# Autodesk Inventor assembly: Robot
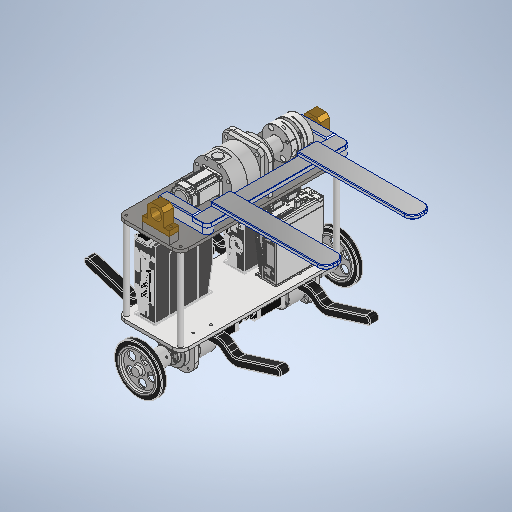
[picture p0: Inventor's stored thumbnail of the model, 512x512]
Saved by Autodesk Inventor 2025.2 (Build 292293000, 293)
## iProperties
Created: 2025-02-20
Part Number: Robot
Document SubType Name: Assembly
Designer: Sergio Quintero
Author: Sergio Quintero
## Documents named in this file (19)
- C:\Users\Sergio Quintero\OneDrive - Universidad Nacional de Colombia\Keio University\Thesis\CAD\Current\Robot.iam
- C:\Users\Sergio Quintero\OneDrive - Universidad Nacional de Colombia\Keio University\Thesis\CAD\Current\Bottom_plate.ipt
- C:\Users\Sergio Quintero\OneDrive - Universidad Nacional de Colombia\Keio University\Thesis\CAD\Current\Top_plate.ipt
- C:\Users\Sergio Quintero\OneDrive - Universidad Nacional de Colombia\Keio University\Thesis\CAD\Current\Structure_bar.ipt
- C:\Users\Sergio Quintero\OneDrive - Universidad Nacional de Colombia\Keio University\Thesis\CAD\Current\Pillow_support.ipt
- C:\Users\Sergio Quintero\OneDrive - Universidad Nacional de Colombia\Keio University\Thesis\CAD\Current\Pillow_block.ipt
- C:\Users\Sergio Quintero\OneDrive - Universidad Nacional de Colombia\Keio University\Thesis\CAD\Current\Gear_support.ipt
- C:\Users\Sergio Quintero\OneDrive - Universidad Nacional de Colombia\Keio University\Thesis\CAD\Current\HPG-32A-33-J2NELA.iam
- C:\Users\Sergio Quintero\OneDrive - Universidad Nacional de Colombia\Keio University\Thesis\CAD\Current\SFC-090SA2-25B-40B.ipt
- C:\Users\Sergio Quintero\OneDrive - Universidad Nacional de Colombia\Keio University\Thesis\CAD\Current\Fork.ipt
- C:\Users\Sergio Quintero\OneDrive - Universidad Nacional de Colombia\Keio University\Thesis\CAD\Current\Gear_support_wheel.ipt
- C:\Users\Sergio Quintero\OneDrive - Universidad Nacional de Colombia\Keio University\Thesis\CAD\Current\HPG-20A-11-J6GDK.iam
- C:\Users\Sergio Quintero\OneDrive - Universidad Nacional de Colombia\Keio University\Thesis\CAD\Current\MRG-50-25-25.ipt
- C:\Users\Sergio Quintero\OneDrive - Universidad Nacional de Colombia\Keio University\Thesis\CAD\Current\Wheel.ipt
- C:\Users\Sergio Quintero\OneDrive - Universidad Nacional de Colombia\Keio University\Thesis\CAD\Current\R88M_K40030S.ipt
- C:\Users\Sergio Quintero\OneDrive - Universidad Nacional de Colombia\Keio University\Thesis\CAD\Current\R88M_1M40030S_S2.ipt
- C:\Users\Sergio Quintero\OneDrive - Universidad Nacional de Colombia\Keio University\Thesis\CAD\Current\Robot_support.ipt
- C:\Users\Sergio Quintero\OneDrive - Universidad Nacional de Colombia\Keio University\Thesis\CAD\Current\R88D_1SN04L_ECT\R88D_1SN04L_ECT.iam
- C:\Users\Sergio Quintero\OneDrive - Universidad Nacional de Colombia\Keio University\Thesis\CAD\Current\R88D_KN04L_ECT\R88D_KN04L_ECT.iam
## Components (32 placed, 18 different names)
1. Bottom_plate:1 — Rigid:1, Rigid:2, Rigid:3, Rigid:4, Rigid:5, Rigid:13, Rigid:14, Angle:1, Rigid:23, Rigid:24, Rigid:25, Rigid:26, Rigid:27, Rigid:28, Rigid:29
2. Top_plate:1 — Rigid:5, Rigid:6, Rigid:8, Rigid:10
3. Structure_bar:1 — Rigid:4
4. Structure_bar:2 — Rigid:3
5. Structure_bar:3 — Rigid:2
6. Structure_bar:4 — Rigid:1
7. Pillow_support:1 — Rigid:6, Rigid:7
8. Pillow_block:1 — Rigid:7
9. Pillow_block:2 — Rigid:9, Rotational:1
10. Pillow_support:2 — Rigid:8, Rigid:9
11. Gear_support:1 — Rigid:10, Rigid:11
12. HPG-32A-33-J2NELA:1 [sub-assembly] — Rigid:11, Rigid:12, Rigid:21
13. SFC-090SA2-25B-40B:1 — Rigid:12
14. Fork:1 — Rotational:1
15. Gear_support_wheel:1 — Rigid:14, Rigid:15
16. Gear_support_wheel:2 — Rigid:13, Rigid:16
17. HPG-20A-11-J6GDK:1 [sub-assembly] — Rigid:15, Rigid:18, Rotational:2
18. HPG-20A-11-J6GDK:2 [sub-assembly] — Rigid:16, Rigid:17, Rigid:22
19. MRG-50-25-25:1 — Rigid:17, Rigid:20
20. MRG-50-25-25:2 — Rigid:18, Rigid:19
21. Wheel:1 — Rigid:20
22. Wheel:2 — Rigid:19, Tangent:1
23. R88M_K40030S:1 — Rigid:21
24. R88M_1M40030S_S2:1 — Rigid:22
25. R88M_1M40030S_S2:2 — Rotational:2
26. Robot_support:1 — Rigid:23
27. Robot_support:2 — Rigid:24
28. Robot_support:3 — Rigid:25
29. Robot_support:4 — Rigid:26
30. R88D_1SN04L_ECT:1 [sub-assembly] — Rigid:27
31. R88D_1SN04L_ECT:2 [sub-assembly] — Rigid:28
32. R88D_KN04L_ECT:1 [sub-assembly] — Rigid:29
## Relationships (33: WeldJoint 29, RevoluteJoint 2, Angle 1, Tangent 1)
- Rigid:1 [WeldJoint]: Bottom_plate:1 ↔ Structure_bar:4
- Rigid:2 [WeldJoint]: Bottom_plate:1 ↔ Structure_bar:3
- Rigid:3 [WeldJoint]: Bottom_plate:1 ↔ Structure_bar:2
- Rigid:4 [WeldJoint]: Bottom_plate:1 ↔ Structure_bar:1
- Rigid:5 [WeldJoint] (260 mm): Bottom_plate:1 ↔ Top_plate:1
- Rigid:6 [WeldJoint]: Top_plate:1 ↔ Pillow_support:1
- Rigid:7 [WeldJoint]: Pillow_support:1 ↔ Pillow_block:1
- Rigid:8 [WeldJoint]: Top_plate:1 ↔ Pillow_support:2
- Rigid:9 [WeldJoint]: Pillow_block:2 ↔ Pillow_support:2
- Rigid:10 [WeldJoint]: Top_plate:1 ↔ Gear_support:1
- Rigid:11 [WeldJoint]: Gear_support:1 ↔ HPG-32A-33-J2NELA:1
- Rigid:12 [WeldJoint] (50 mm): HPG-32A-33-J2NELA:1 ↔ SFC-090SA2-25B-40B:1
- Rotational:1 [RevoluteJoint] (5 mm): Pillow_block:2 ↔ Fork:1
- Rigid:13 [WeldJoint]: Bottom_plate:1 ↔ Gear_support_wheel:2
- Rigid:14 [WeldJoint]: Bottom_plate:1 ↔ Gear_support_wheel:1
- Rigid:15 [WeldJoint]: Gear_support_wheel:1 ↔ HPG-20A-11-J6GDK:1
- Rigid:16 [WeldJoint]: Gear_support_wheel:2 ↔ HPG-20A-11-J6GDK:2
- Rigid:17 [WeldJoint] (15 mm): HPG-20A-11-J6GDK:2 ↔ MRG-50-25-25:1
- Rigid:18 [WeldJoint] (15 mm): HPG-20A-11-J6GDK:1 ↔ MRG-50-25-25:2
- Rigid:19 [WeldJoint] (3 mm): MRG-50-25-25:2 ↔ Wheel:2
- Rigid:20 [WeldJoint] (3 mm): MRG-50-25-25:1 ↔ Wheel:1
- Rigid:21 [WeldJoint]: HPG-32A-33-J2NELA:1 ↔ R88M_K40030S:1
- Rigid:22 [WeldJoint]: HPG-20A-11-J6GDK:2 ↔ R88M_1M40030S_S2:1
- Rotational:2 [RevoluteJoint]: HPG-20A-11-J6GDK:1 ↔ R88M_1M40030S_S2:2
- Angle:1 (0 deg): Bottom_plate:1
- Tangent:1: Wheel:2
- Rigid:23 [WeldJoint]: Bottom_plate:1 ↔ Robot_support:1
- Rigid:24 [WeldJoint]: Bottom_plate:1 ↔ Robot_support:2
- Rigid:25 [WeldJoint]: Bottom_plate:1 ↔ Robot_support:3
- Rigid:26 [WeldJoint]: Bottom_plate:1 ↔ Robot_support:4
- Rigid:27 [WeldJoint]: Bottom_plate:1 ↔ R88D_1SN04L_ECT:1
- Rigid:28 [WeldJoint]: Bottom_plate:1 ↔ R88D_1SN04L_ECT:2
- Rigid:29 [WeldJoint]: Bottom_plate:1 ↔ R88D_KN04L_ECT:1
